# Autodesk Inventor assembly: gripper assembly
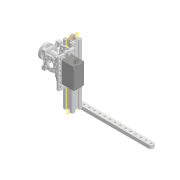
[picture p0: Inventor's stored thumbnail of the model, 180x180]
Saved by Autodesk Inventor 2020 (Build 240168000, 168)
## iProperties
Created: 2020-01-03
Part Number: gripper assembly
Document SubType Name: Assembly
Designer: ball
Author: ball
## Documents named in this file (4)
- C:\FTC\FTC8863CAD\2019 Robot\Collection\gripper assembly.iam
- C:\FTC\FTC8863CAD\Actobotics\565 parts\565026.ipt
- C:\FTC\FTC8863CAD\2019 Robot\Collection\servo block assembly.iam
- C:\FTC\FTC8863CAD\2019 Robot\Collection\grabber arm.ipt
## Components (3 placed, 3 different names)
1. 565026:1 — Mate:1, Mate:2, Mate:3, Flush:1
2. servo block assembly:1 [sub-assembly] — Mate:1, Mate:2, Mate:3, Flush:1
3. grabber arm:1
## Relationships (4: Mate 3, Flush 1)
- Mate:1: 565026:1 ↔ servo block assembly:1
- Mate:2: 565026:1 ↔ servo block assembly:1
- Mate:3: 565026:1 ↔ servo block assembly:1
- Flush:1 (77.216 mm): 565026:1 ↔ servo block assembly:1
